# Autodesk Inventor assembly: v1 1
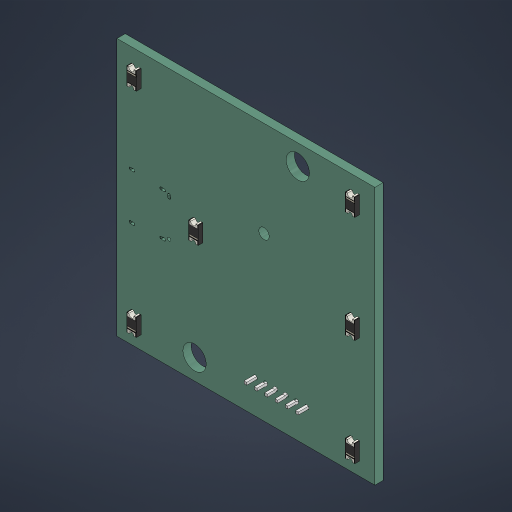
[picture p0: Inventor's stored thumbnail of the model, 512x512]
Saved by Autodesk Inventor 2023 (Build 270158000, 158)
## iProperties
Company: Kicad
Created: 2023-11-20
Part Number: v1 1
Description: KiCad electronic assembly
Document SubType Name: Assembly
Designer: Leon
Authority: Unknown
Sending System: KiCad to STEP converter
Preprocessor: Open CASCADE STEP processor 7.7
Title: v1.step
Author: Pcbnew
## Documents named in this file (8)
- C:\Users\Leon\OneDrive\projekti_2022\24-lampadine\12-pcb\v1\export for inventor\v1-rev1\v1_rev1.iam
- C:\Users\Leon\OneDrive\projekti_2022\24-lampadine\12-pcb\v1\export for inventor\v1-rev1\D_1206_3216Metric.iam
- C:\Users\Leon\OneDrive\projekti_2022\24-lampadine\12-pcb\v1\export for inventor\v1-rev1\C_0201_0603Metric.iam
- C:\Users\Leon\OneDrive\projekti_2022\24-lampadine\12-pcb\v1\export for inventor\v1-rev1\R_0603_1608Metric.iam
- C:\Users\Leon\OneDrive\projekti_2022\24-lampadine\12-pcb\v1\export for inventor\v1-rev1\TSOT-23.iam
- C:\Users\Leon\OneDrive\projekti_2022\24-lampadine\12-pcb\v1\export for inventor\v1-rev1\v1 PCB.ipt
- C:\Users\Leon\OneDrive\projekti_2022\24-lampadine\99-foreign parts\usb_c_12401610E4#2A.ipt
- C:\Users\Leon\OneDrive\projekti_2022\24-lampadine\99-foreign parts\molex_angle_532540670.ipt
## Components (23 placed, 23 different names)
1. 2 [sub-assembly]
2. 3 [sub-assembly]
3. 4 [sub-assembly]
4. 5 [sub-assembly]
5. 6 [sub-assembly]
6. 7 [sub-assembly]
7. 9 [sub-assembly]
8. 11 [sub-assembly]
9. 12 [sub-assembly]
10. 13 [sub-assembly]
11. 14 [sub-assembly]
12. 15 [sub-assembly]
13. 16 [sub-assembly]
14. 17 [sub-assembly]
15. 18 [sub-assembly]
16. 19 [sub-assembly]
17. 20 [sub-assembly]
18. 22 [sub-assembly]
19. 23 [sub-assembly]
20. 24 [sub-assembly]
21. 25 — Rigid:1, Mate:1, Flush:1, Flush:2
22. usb_c_12401610E4#2A:1 — Rigid:1
23. molex_angle_532540670:1 — Mate:1, Flush:1, Flush:2
## Relationships (4: Flush 2, WeldJoint 1, Mate 1)
- Rigid:1 [WeldJoint]: 25 ↔ usb_c_12401610E4#2A:1
- Mate:1: 25 ↔ molex_angle_532540670:1
- Flush:1 (0.5 mm): 25 ↔ molex_angle_532540670:1
- Flush:2 (11.2 mm): 25 ↔ molex_angle_532540670:1
